# Autodesk Inventor assembly: Vert
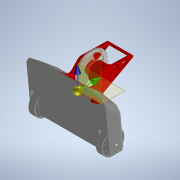
[picture p0: Inventor's stored thumbnail of the model, 180x180]
Saved by Autodesk Inventor 2020 (Build 240168000, 168)
## iProperties
Created: 2024-01-30
Part Number: Vert
Document SubType Name: Assembly
Designer: smz3rm
Mass: 418.507 g
Surface Area: 1611.45 cm^2
Volume: 310.377 cm^3
Density: 1.34838 g/cm^3
Author: smz3rm
## Documents named in this file (13)
- C:\Users\smz3rm\OneDrive - BP\Documents\Battlebots\VerticalSpinner\Vert.iam
- C:\Users\smz3rm\OneDrive - BP\Documents\Battlebots\VerticalSpinner\RepeatDriveBrushedMk2 - 4mm.iam
- C:\Users\smz3rm\OneDrive - BP\Documents\Battlebots\Switch.ipt
- C:\Users\smz3rm\OneDrive - BP\Documents\Battlebots\SwitchHolder.ipt
- C:\Users\smz3rm\OneDrive - BP\Documents\Battlebots\FS2A.ipt
- C:\Users\smz3rm\OneDrive - BP\Documents\Battlebots\BatteryV1.ipt
- C:\Users\smz3rm\OneDrive - BP\Documents\Battlebots\WeaponBearingV1.ipt
- C:\Users\smz3rm\OneDrive - BP\Documents\Battlebots\WeaponMotorV1.ipt
- C:\Users\smz3rm\OneDrive - BP\Documents\Battlebots\WeaponV2.ipt
- C:\Users\smz3rm\OneDrive - BP\Documents\Battlebots\VerticalSpinner\VertBody.ipt
- C:\Users\smz3rm\OneDrive - BP\Documents\Battlebots\VerticalSpinner\VertWheelV1.ipt
- C:\Users\smz3rm\OneDrive - BP\Documents\Battlebots\BladeHubV1.ipt
- C:\Users\smz3rm\OneDrive - BP\Documents\Battlebots\VerticalSpinner\VertWeaponMount.iam
## Components (14 placed, 12 different names)
1. RepeatDriveBrushedMk2 - 4mm:1 [sub-assembly] — Mate:7, Mate:8, Mate:28, Mate:29
2. RepeatDriveBrushedMk2 - 4mm:2 [sub-assembly] — Mate:3, Mate:5, Mate:6, Mate:27
3. Switch:1 — Mate:23, Mate:24, Mate:25
4. SwitchHolder:1 — Mate:23, Mate:24, Mate:25, Mate:26
5. FS2A:1
6. BatteryV1:1 — Mate:22
7. WeaponBearingV1:1 — Mate:17, Flush:2
8. WeaponMotorV1:1 — Mate:9, Mate:10, Mate:12, Tangent:2, MotorFlushTemp, Mate:18, Mate:19, Mate:20, Mate:21
9. WeaponV2:1 — Mate:9, Mate:11
10. VertBody:1 — Mate:3, Mate:13, Flush:1, Mate:14, Mate:22, Mate:26, Mate:27, Mate:28, Mate:29, Mate:30, Mate:31, Mate:32, Mate:33, Mate:34, Mate:35
11. VertWheelV1:1 — Mate:7, Mate:8
12. VertWheelV1:2 — Mate:5, Mate:6
13. BladeHubV1:1 — Mate:10, Mate:11, Mate:12, Tangent:2
14. VertWeaponMount:1 [sub-assembly] — Mate:13, Flush:1, Mate:14, MotorFlushTemp, Mate:17, Flush:2, Mate:18, Mate:19, Mate:20, Mate:21, Mate:30, Mate:31, Mate:32, Mate:33, Mate:34, Mate:35
## Relationships (34: Mate 31, Flush 2, Tangent 1)
- Mate:3: RepeatDriveBrushedMk2 - 4mm:2 ↔ VertBody:1
- Mate:5: RepeatDriveBrushedMk2 - 4mm:2 ↔ VertWheelV1:2
- Mate:6 (1 mm): RepeatDriveBrushedMk2 - 4mm:2 ↔ VertWheelV1:2
- Mate:7: RepeatDriveBrushedMk2 - 4mm:1 ↔ VertWheelV1:1
- Mate:8 (1 mm): RepeatDriveBrushedMk2 - 4mm:1 ↔ VertWheelV1:1
- Mate:9: WeaponMotorV1:1 ↔ WeaponV2:1
- Mate:10: WeaponMotorV1:1 ↔ BladeHubV1:1
- Mate:11: WeaponV2:1 ↔ BladeHubV1:1
- Mate:12: WeaponMotorV1:1 ↔ BladeHubV1:1
- Tangent:2: WeaponMotorV1:1 ↔ BladeHubV1:1
- Mate:13: VertBody:1 ↔ VertWeaponMount:1
- Flush:1: VertBody:1 ↔ VertWeaponMount:1
- Mate:14 (0.4 mm): VertBody:1 ↔ VertWeaponMount:1
- MotorFlushTemp [Mate]: WeaponMotorV1:1 ↔ VertWeaponMount:1
- Mate:17: WeaponBearingV1:1 ↔ VertWeaponMount:1
- Flush:2: WeaponBearingV1:1 ↔ VertWeaponMount:1
- Mate:18: WeaponMotorV1:1 ↔ VertWeaponMount:1
- Mate:19: WeaponMotorV1:1 ↔ VertWeaponMount:1
- Mate:20: WeaponMotorV1:1 ↔ VertWeaponMount:1
- Mate:21: WeaponMotorV1:1 ↔ VertWeaponMount:1
- Mate:22: BatteryV1:1 ↔ VertBody:1
- Mate:23: Switch:1 ↔ SwitchHolder:1
- Mate:24: Switch:1 ↔ SwitchHolder:1
- Mate:25: Switch:1 ↔ SwitchHolder:1
- Mate:26: SwitchHolder:1 ↔ VertBody:1
- Mate:27: RepeatDriveBrushedMk2 - 4mm:2 ↔ VertBody:1
- Mate:28: RepeatDriveBrushedMk2 - 4mm:1 ↔ VertBody:1
- Mate:29: RepeatDriveBrushedMk2 - 4mm:1 ↔ VertBody:1
- Mate:30: VertBody:1 ↔ VertWeaponMount:1
- Mate:31: VertBody:1 ↔ VertWeaponMount:1
- Mate:32: VertBody:1 ↔ VertWeaponMount:1
- Mate:33: VertBody:1 ↔ VertWeaponMount:1
- Mate:34: VertBody:1 ↔ VertWeaponMount:1
- Mate:35: VertBody:1 ↔ VertWeaponMount:1
## Named parameters: WeaponMountTolerance = 0.4 mm
